# Autodesk Inventor assembly: cover2
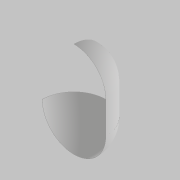
[picture p0: Inventor's stored thumbnail of the model, 180x180]
Saved by Autodesk Inventor 2021 (Build 250183000, 183)
## iProperties
Created: 2021-06-01
Part Number: cover2
Document SubType Name: Assembly
Designer: Watchdog
Author: Watchdog
## Documents named in this file (4)
- C:\Users\Watchdog\OneDrive - Flinders\Advn Mech Design Shared\6_Development\2_Design\inventor\cover\cover2.iam
- C:\Users\Watchdog\OneDrive - Flinders\Advn Mech Design Shared\6_Development\2_Design\inventor\cover\cover2_cap.ipt
- C:\Users\Watchdog\OneDrive - Flinders\Advn Mech Design Shared\6_Development\2_Design\inventor\cover\cover2_sule.ipt
- C:\Users\Watchdog\OneDrive - Flinders\Advn Mech Design Shared\6_Development\2_Design\inventor\cover\cover2_sule_inner.ipt
## Components (3 placed, 3 different names)
1. cover2_cap:1 — Flush:1, Mate:4, Flush:2, Mate:6
2. cover2_sule:1 — Mate:1, Mate:2, Mate:3, Flush:1, Mate:4, Flush:2, Angle:1, Mate:5
3. cover2_sule_inner:1 — Angle:1, Mate:5, Mate:6
## Relationships (9: Mate 6, Flush 2, Angle 1)
- Mate:1: cover2_sule:1
- Mate:2: cover2_sule:1
- Mate:3: cover2_sule:1
- Flush:1: cover2_cap:1 ↔ cover2_sule:1
- Mate:4: cover2_cap:1 ↔ cover2_sule:1
- Flush:2: cover2_cap:1 ↔ cover2_sule:1
- Angle:1 (0 deg): cover2_sule:1 ↔ cover2_sule_inner:1
- Mate:5: cover2_sule:1 ↔ cover2_sule_inner:1
- Mate:6: cover2_cap:1 ↔ cover2_sule_inner:1
